# Autodesk Inventor assembly: Sumiriki
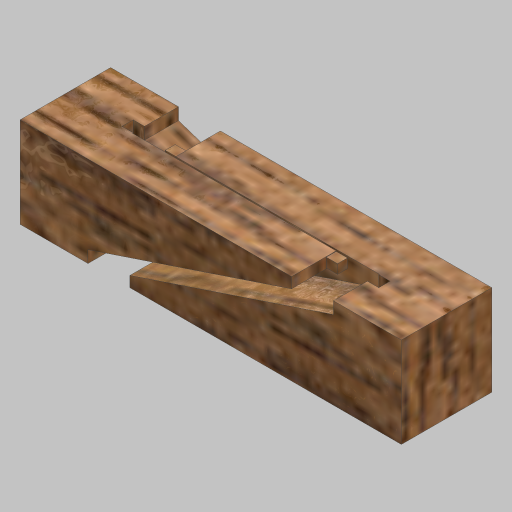
[picture p0: Inventor's stored thumbnail of the model, 512x512]
Saved by Autodesk Inventor 2023 (Build 270158000, 158)
## iProperties
Created: 2026-07-03
Part Number: Sumiriki
Document SubType Name: Assembly
Designer: MARTIN MAESTRE
Author: MARTIN MAESTRE
## Documents named in this file (2)
- C:\Users\MARTIN MAESTRE\OneDrive - Universidad de los Andes\POSTGRADO\202610\MAESTRIA\PROBLEMA ESPECIAL\CADS_TOLERANCIAS\Repositorio\Sumiriki Isuka Tsugi\Sumiriki.iam
- C:\Users\MARTIN MAESTRE\OneDrive - Universidad de los Andes\POSTGRADO\202610\MAESTRIA\PROBLEMA ESPECIAL\CADS_TOLERANCIAS\Repositorio\Sumiriki Isuka Tsugi\Sumiriki_half.ipt
## Components (2 placed, 1 different names)
1. Sumiriki_half:1 — Nivelación:1, Coincidencia:1, Coincidencia:2, Nivelación:2, Nivelación:3
2. Sumiriki_half:2 — Nivelación:2, Nivelación:3
## Relationships (5: Flush 3, Mate 2)
- Nivelación:1 [Flush]: Sumiriki_half:1
- Coincidencia:1 [Mate]: Sumiriki_half:1
- Coincidencia:2 [Mate]: Sumiriki_half:1
- Nivelación:2 [Flush]: Sumiriki_half:1 ↔ Sumiriki_half:2
- Nivelación:3 [Flush]: Sumiriki_half:1 ↔ Sumiriki_half:2
